# Autodesk Inventor assembly: gpio
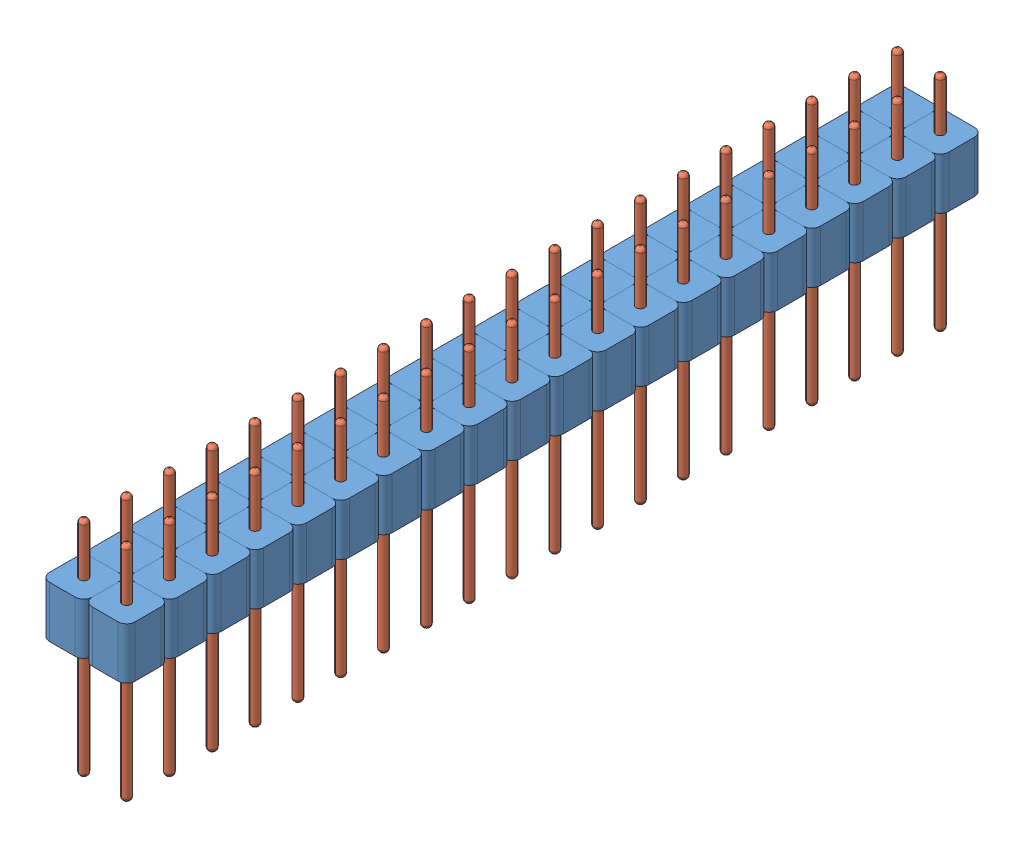
[picture p0: shaded view drawn from the part files that the assembly names]
Saved by Autodesk Inventor 2015 (Build 190159000, 159)
## iProperties
Created: 2015-12-03
Part Number: gpio
Document SubType Name: Assembly
Designer: david
Author: david
## Documents named in this file (3)
- Z:\gip\Inventor\generatie 7\Frame\Electronica\raspberry pi\gpio.iam
- Z:\gip\Inventor\generatie 7\Frame\Electronica\raspberry pi\pin.ipt
- Z:\gip\Inventor\generatie 7\Frame\Electronica\raspberry pi\block.ipt
## Components (80 placed, 2 different names)
1. block:1 — Mate:1, Flush:1
2. pin:1 — Mate:1, Flush:1
3. block:2
4. pin:2
5. block:3
6. pin:3
7. block:4
8. pin:4
9. block:5
10. pin:5
11. block:6
12. pin:6
13. block:7
14. pin:7
15. block:8
16. pin:8
17. block:9
18. pin:9
19. block:10
20. pin:10
21. block:11
22. pin:11
23. block:12
24. pin:12
25. block:13
26. pin:13
27. block:14
28. pin:14
29. block:15
30. pin:15
31. block:16
32. pin:16
33. block:17
34. pin:17
35. block:18
36. pin:18
37. block:19
38. pin:19
39. block:20
40. pin:20
41. block:21
42. pin:21
43. block:22
44. pin:22
45. block:23
46. pin:23
47. block:24
48. pin:24
49. block:25
50. pin:25
51. block:26
52. pin:26
53. block:27
54. pin:27
55. block:28
56. pin:28
57. block:29
58. pin:29
59. block:30
60. pin:30
61. block:31
62. pin:31
63. block:32
64. pin:32
65. block:33
66. pin:33
67. block:34
68. pin:34
69. block:35
70. pin:35
71. block:36
72. pin:36
73. block:37
74. pin:37
75. block:38
76. pin:38
77. block:39
78. pin:39
79. block:40
80. pin:40
## Component patterns: (40 elements, first: block:1 + pin:1)
## Relationships (2: Mate 1, Flush 1)
- Mate:1: block:1 ↔ pin:1
- Flush:1 (3 mm): block:1 ↔ pin:1
